# Autodesk Inventor assembly: Asem
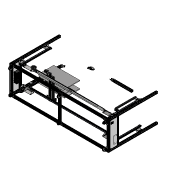
[picture p0: Inventor's stored thumbnail of the model, 180x180]
Saved by Autodesk Inventor 2020 (Build 240168000, 168)
## iProperties
Created: 2021-02-24
Part Number: Asem
Document SubType Name: Assembly
Designer: magnarecta
Author: magnarecta
## Documents named in this file (7)
- D:\Documents\GitHub\Eto_Project\Hardware\Asem\Asem.iam
- D:\Documents\GitHub\Eto_Project\Hardware\Parts\MISUMI_FRAMES\artschallenge2022c.iam
- D:\Documents\GitHub\Eto_Project\Hardware\Asem\CCM_Unit.iam
- D:\Documents\GitHub\Eto_Project\Hardware\Asem\Display_Unit.iam
- D:\Documents\GitHub\Eto_Project\Hardware\Parts\Grabcad\nema-23-stepper-motors-driver-1.snapshot.7\DM542T Digital Stepper Drive.ipt
- D:\Documents\GitHub\Eto_Project\Hardware\Parts\Grabcad\mean-well-lrs-350-24-1.snapshot.3\meanwell_lrs-350-24_UPDATED.ipt
- D:\Documents\GitHub\Eto_Project\Hardware\Parts\Grabcad\ac-power-switch-assembly-1.snapshot.2\AC Power Switch Assy.iam
## Components (13 placed, 6 different names)
1. artschallenge2022c:1 [sub-assembly] — フラッシュ:1, 角度:1, メイト:1, フラッシュ:2, 角度:2, メイト:4, 角度:3, メイト:5, メイト:6, メイト:7, フラッシュ:4
2. CCM_Unit:1 [sub-assembly] — フラッシュ:1, 角度:1, メイト:1, フラッシュ:2, 挿入:1, 挿入:2, フラッシュ:4
3. Display_Unit:1 [sub-assembly] — 挿入:1, 挿入:2
4. meanwell_lrs-350-24_UPDATED:1 — メイト:4, 角度:3
5. AC Power Switch Assy:1 [sub-assembly] — メイト:6, フラッシュ:3
6. AC Power Switch Assy:2 [sub-assembly] — メイト:7, フラッシュ:3
7. DM542T Digital Stepper Drive:1
8. DM542T Digital Stepper Drive:2
9. DM542T Digital Stepper Drive:3
10. DM542T Digital Stepper Drive:4
11. DM542T Digital Stepper Drive:5
12. DM542T Digital Stepper Drive:6
13. DM542T Digital Stepper Drive:7 — 角度:2, メイト:5
## Component patterns: (7 elements, first: DM542T Digital Stepper Drive:1)
## Relationships (14: Mate 5, Flush 4, Angle 3, Insert 2)
- フラッシュ:1 [Flush] (60 mm): artschallenge2022c:1 ↔ CCM_Unit:1
- 角度:1 [Angle] (180 deg): artschallenge2022c:1 ↔ CCM_Unit:1
- メイト:1 [Mate]: artschallenge2022c:1 ↔ CCM_Unit:1
- フラッシュ:2 [Flush]: artschallenge2022c:1 ↔ CCM_Unit:1
- 挿入:1 [Insert]: CCM_Unit:1 ↔ Display_Unit:1
- 角度:2 [Angle] (90 deg): artschallenge2022c:1 ↔ DM542T Digital Stepper Drive:7
- メイト:4 [Mate]: artschallenge2022c:1 ↔ meanwell_lrs-350-24_UPDATED:1
- 角度:3 [Angle] (90 deg): artschallenge2022c:1 ↔ meanwell_lrs-350-24_UPDATED:1
- メイト:5 [Mate]: artschallenge2022c:1 ↔ DM542T Digital Stepper Drive:7
- メイト:6 [Mate]: artschallenge2022c:1 ↔ AC Power Switch Assy:1
- メイト:7 [Mate]: artschallenge2022c:1 ↔ AC Power Switch Assy:2
- フラッシュ:3 [Flush]: AC Power Switch Assy:1 ↔ AC Power Switch Assy:2
- 挿入:2 [Insert]: CCM_Unit:1 ↔ Display_Unit:1
- フラッシュ:4 [Flush]: artschallenge2022c:1 ↔ CCM_Unit:1
